# Autodesk Inventor assembly: Sestava_krabicka
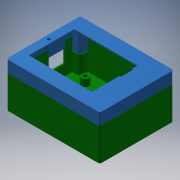
[picture p0: Inventor's stored thumbnail of the model, 180x180]
Saved by Autodesk Inventor 2019 (Build 230136000, 136)
## iProperties
Created: 2019-03-26
Part Number: Sestava_krabicka
Document SubType Name: Assembly
Designer: janza
Author: janza
## Documents named in this file (3)
- D:\Users\janza\Google Disk\Documents\FEL ČVUT\BP_PROJ\piskvorky_case\client_ArdEthernet_case\Sestava_krabicka.iam
- D:\Users\janza\Google Disk\Documents\FEL ČVUT\BP_PROJ\piskvorky_case\client_ArdEthernet_case\case_bottom.ipt
- D:\Users\janza\Google Disk\Documents\FEL ČVUT\BP_PROJ\piskvorky_case\client_ArdEthernet_case\case_top.ipt
## Components (2 placed, 2 different names)
1. case_bottom:1 — Mate:1, Flush:1, Flush:2
2. case_top:1 — Mate:1, Flush:1, Flush:2
## Relationships (3: Flush 2, Mate 1)
- Mate:1: case_bottom:1 ↔ case_top:1
- Flush:1: case_bottom:1 ↔ case_top:1
- Flush:2: case_bottom:1 ↔ case_top:1
